# Autodesk Inventor assembly: Assembly1
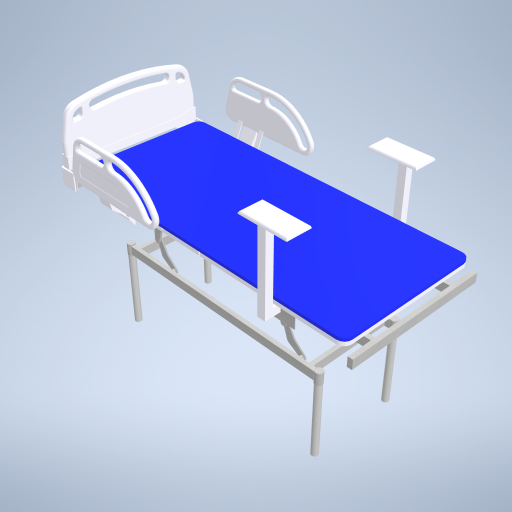
[picture p0: Inventor's stored thumbnail of the model, 512x512]
Saved by Autodesk Inventor 2023 (Build 270158000, 158)
## iProperties
Created: 2023-02-13
Part Number: Assembly1
Document SubType Name: Assembly
Designer: klebe
Author: klebe
## Documents named in this file (2)
- C:\Users\klebe\OneDrive\Documents\GitHub\Sala-braquiterapia\Sala de Braquiterapia\Inventor\hospital-bed-ranjang-pasien-tempat-tidur-pasien-1.snapshot.4\Assembly1.iam
- C:\Users\klebe\OneDrive\Documents\GitHub\Sala-braquiterapia\Sala de Braquiterapia\Inventor\hospital-bed-ranjang-pasien-tempat-tidur-pasien-1.snapshot.4\cama\camaAssem1-RP1.iam
## Components (1 placed, 1 different names)
1. camaAssem1-RP1:1 [sub-assembly] — Mate:1, Mate:2
## Relationships (2: Mate 2)
- Mate:1: camaAssem1-RP1:1
- Mate:2: camaAssem1-RP1:1
